# Autodesk Inventor assembly: axis_module_old
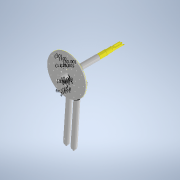
[picture p0: Inventor's stored thumbnail of the model, 180x180]
Saved by Autodesk Inventor 2021 (Build 250183000, 183)
## iProperties
Created: 2021-02-07
Part Number: axis_module_old
Document SubType Name: Assembly
Designer: dsdan
Author: dsdan
## Documents named in this file (8)
- E:\OneDrive - Imperial College London\DragonVision_DanielKo\Instrumentation\Ephys_rig_2021\axis_module_old.iam
- E:\OneDrive - Imperial College London\DragonVision_DanielKo\Instrumentation\Ephys_rig_2021\Imported Components\PH30_M-Solidworks.ipt
- E:\OneDrive - Imperial College London\DragonVision_DanielKo\Instrumentation\Ephys_rig_2021\Imported Components\TR100_M-Solidworks.ipt
- E:\OneDrive - Imperial College London\DragonVision_DanielKo\Instrumentation\Ephys_rig_2021\Holder\body_adjustable_parametric.ipt
- E:\OneDrive - Imperial College London\DragonVision_DanielKo\Instrumentation\Ephys_rig_2021\Imported Components\RA180_M-Solidworks.ipt
- E:\OneDrive - Imperial College London\DragonVision_DanielKo\Instrumentation\Ephys_rig_2021\Imported Components\TR150_M-Solidworks\TR150_M-Solidworks.ipt
- E:\OneDrive - Imperial College London\DragonVision_DanielKo\Instrumentation\Ephys_rig_2021\tool_adapter_2.ipt
- E:\OneDrive - Imperial College London\DragonVision_DanielKo\Instrumentation\Ephys_rig_2021\baseplate.ipt
## Components (9 placed, 7 different names)
1. PH30_M-Solidworks:1 — Mate:33, Rotation:7, Mate:41
2. TR100_M-Solidworks:1 — Mate:5, Mate:6, Mate:42
3. body_adjustable_parametric:1 — Mate:5, Mate:6, Rotation:6
4. RA180_M-Solidworks:3 — Mate:31, Mate:38, Mate:40, Mate:46
5. RA180_M-Solidworks:4 — Mate:36, Mate:39, Mate:43
6. TR150_M-Solidworks:2 — Mate:31, Mate:45
7. tool_adapter_2:1 — Mate:32, Mate:34, Mate:35, Mate:36, Mate:38, Mate:39, Mate:40, Mate:44, Mate:45, Mate:46
8. baseplate:1 — Mate:32, Mate:33, Mate:34, Mate:35, Rotation:7, Mate:41, Flush:3, Rotation:6
9. TR150_M-Solidworks:3 — Mate:43, Mate:44
## Relationships (21: Mate 18, RelateRotation 2, Flush 1)
- [Mate]: PH30_M-Solidworks:1 ↔ TR100_M-Solidworks:1
- Mate:5: TR100_M-Solidworks:1 ↔ body_adjustable_parametric:1
- Mate:6: TR100_M-Solidworks:1 ↔ body_adjustable_parametric:1
- Mate:31: RA180_M-Solidworks:3 ↔ TR150_M-Solidworks:2
- Mate:32: tool_adapter_2:1 ↔ baseplate:1
- Mate:33: PH30_M-Solidworks:1 ↔ baseplate:1
- Mate:34: tool_adapter_2:1 ↔ baseplate:1
- Mate:35: tool_adapter_2:1 ↔ baseplate:1
- Rotation:6 [RelateRotation] (1 ul): body_adjustable_parametric:1 ↔ baseplate:1
- Rotation:7 [RelateRotation] (-1 ul): PH30_M-Solidworks:1 ↔ baseplate:1
- Mate:36: RA180_M-Solidworks:4 ↔ tool_adapter_2:1
- Mate:38: RA180_M-Solidworks:3 ↔ tool_adapter_2:1
- Mate:39: RA180_M-Solidworks:4 ↔ tool_adapter_2:1
- Mate:40: RA180_M-Solidworks:3 ↔ tool_adapter_2:1
- Mate:41: PH30_M-Solidworks:1 ↔ baseplate:1
- Flush:3: baseplate:1
- Mate:42: TR100_M-Solidworks:1
- Mate:43: RA180_M-Solidworks:4 ↔ TR150_M-Solidworks:3
- Mate:44: tool_adapter_2:1 ↔ TR150_M-Solidworks:3
- Mate:45: TR150_M-Solidworks:2 ↔ tool_adapter_2:1
- Mate:46: RA180_M-Solidworks:3 ↔ tool_adapter_2:1
